# Autodesk Inventor assembly: TL_50_40
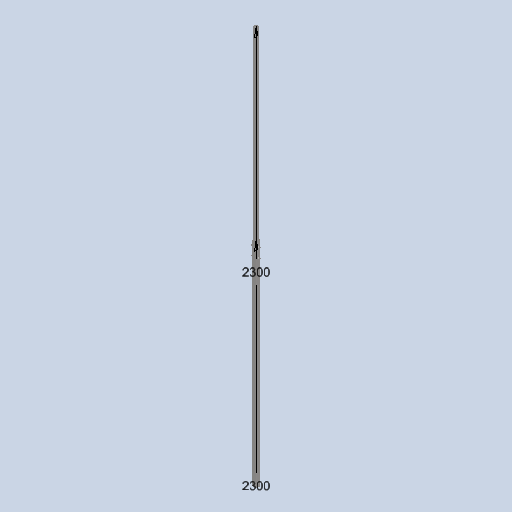
[picture p0: Inventor's stored thumbnail of the model, 512x512]
Saved by Autodesk Inventor 2023 (Build 270158000, 158)
## iProperties
Created: 2025-04-11
Part Number: TL_50_40
Document SubType Name: Assembly
Designer: NELLY NDUNG'U
Author: NELLY NDUNG'U
## Documents named in this file (5)
- N:\NAKUJA\CAD FILES\AIRFRAME\LP003\TL_50_40.iam
- N:\NAKUJA\CAD FILES\AIRFRAME\LP003\TL_40.iam
- N:\NAKUJA\CAD FILES\AIRFRAME\LP003\TL_50.iam
- C:\Users\User\Documents\Inventor\Content Center Files\R2023\en-US\ANSI B18.2.3.5M\ANSI B18.2.3.5M - M16 x 2 x 65.ipt
- C:\Users\User\Documents\Inventor\Content Center Files\R2023\en-US\ANSI B 18.2.4.1 M(1)\ANSI B 18.2.4.1 M - M16 x 2Style 1.ipt
## Components (6 placed, 4 different names)
1. TL_40:1 [sub-assembly] — Mate:1, Mate:2, Mate:3
2. TL_50:1 [sub-assembly] — Mate:1, Mate:2, Mate:3, Insert:1, Insert:2, Insert:3, Insert:4
3. Hex Bolt - Metric M16 x 2 x 65:1 — Insert:1
4. Hex Bolt - Metric M16 x 2 x 65:2 — Insert:2
5. Hex Nut Metric M16 x 2:1 — Insert:3
6. Hex Nut Metric M16 x 2:2 — Insert:4
## Relationships (7: Insert 4, Mate 3)
- Mate:1 (1 mm): TL_40:1 ↔ TL_50:1
- Mate:2 (1 mm): TL_40:1 ↔ TL_50:1
- Mate:3 (-300 mm): TL_40:1 ↔ TL_50:1
- Insert:1: TL_50:1 ↔ Hex Bolt - Metric M16 x 2 x 65:1
- Insert:2: TL_50:1 ↔ Hex Bolt - Metric M16 x 2 x 65:2
- Insert:3: TL_50:1 ↔ Hex Nut Metric M16 x 2:1
- Insert:4: TL_50:1 ↔ Hex Nut Metric M16 x 2:2
